# Autodesk Inventor assembly: Wheel_MIR
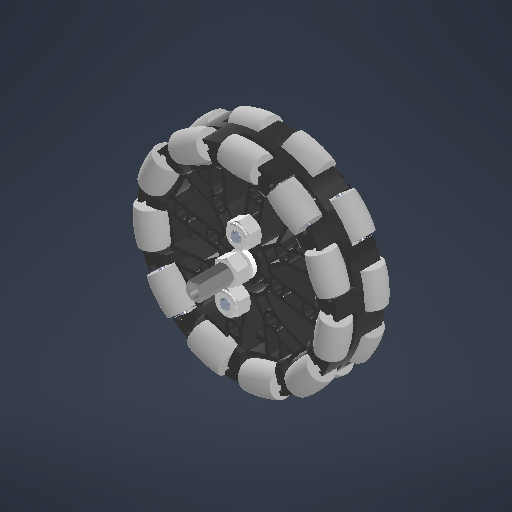
[picture p0: Inventor's stored thumbnail of the model, 512x512]
Saved by Autodesk Inventor 2026.1 (Build 301233000, 233)
## iProperties
Created: 2025-08-03
Part Number: Wheel_MIR
Document SubType Name: Assembly
Designer: roejo
Author: roejo
## Documents named in this file (12)
- C:\Users\roejo\OneDrive\Documents\2026WorldChampionRobot\Robots\Worlds\Subassemblies\Wheel_MIR.iam
- C:\Users\roejo\OneDrive\Documents\2026WorldChampionRobot\Library\Custom Parts\HS 48T Gear, No Insert, Lathe_MIR.iam
- C:\Users\roejo\OneDrive\Documents\2026WorldChampionRobot\Library\VEX-CAD-Inventor-1.4.2\Motion\Spacers\Washer Teflon\TWasher .375 OD x .06250.ipt
- C:\Users\roejo\OneDrive\Documents\2026WorldChampionRobot\Library\VEX-CAD-Inventor-1.4.2\Motion\Spacers\Washer Teflon.ipt
- C:\Users\roejo\OneDrive\Documents\2026WorldChampionRobot\Library\VEX-CAD-Inventor-1.4.2\Structure\Hardware\alu_nylock_MIR.ipt
- C:\Users\roejo\OneDrive\Documents\2026WorldChampionRobot\Library\VEX-CAD-Inventor-1.4.2\Structure\Standoff\Standoff .50.ipt
- C:\Users\roejo\OneDrive\Documents\2026WorldChampionRobot\Library\VEX-CAD-Inventor-1.4.2\Structure\Standoff.ipt
- C:\Users\roejo\OneDrive\Documents\2026WorldChampionRobot\Library\VEX-CAD-Inventor-1.4.2\Structure\Hardware\Screw Steel - Star\SScrew Star Smooth 1.250.ipt
- C:\Users\roejo\OneDrive\Documents\2026WorldChampionRobot\Library\VEX-CAD-Inventor-1.4.2\Structure\Hardware\Screw Steel - Star.ipt
- C:\Users\roejo\OneDrive\Documents\2026WorldChampionRobot\Library\VEX-CAD-Inventor-1.4.2\Motion\Wheels\Omni Wheel\3.25 Omni AS, No Insert_MIR.iam
- C:\Users\roejo\OneDrive\Documents\2026WorldChampionRobot\Library\VEX-CAD-Inventor-1.4.2\Structure\Hardware\Nut Nylon\Nut Nylon - Black.ipt
- C:\Users\roejo\OneDrive\Documents\2026WorldChampionRobot\Library\VEX-CAD-Inventor-1.4.2\Structure\Hardware\Nut Nylon.ipt
## Components (10 placed, 7 different names)
1. HS 48T Gear, No Insert, Lathe_MIR:1 [sub-assembly] — Insert:11, Insert:13, Insert:15, Insert:14, Insert:11
2. TWasher .375 OD x .06250:1 — Insert:5, Insert:18
3. alu_nylock_MIR:1 — Insert:5, Insert:6
4. Standoff .50:1 — Insert:6
5. alu_nylock_MIR:2 — Insert:17
6. SScrew Star Smooth 1.250:1 — Insert:11
7. alu_nylock_MIR:3 — Insert:16
8. SScrew Star Smooth 1.250:2 — Insert:13
9. 3.25 Omni AS, No Insert_MIR:1 [sub-assembly] — Insert:18, Insert:17, Insert:16, Insert:15, Insert:14
10. Nut Nylon - Black:1 — Insert:11
## Relationships (10: Insert 10)
- Insert:5: TWasher .375 OD x .06250:1 ↔ alu_nylock_MIR:1
- Insert:6: alu_nylock_MIR:1 ↔ Standoff .50:1
- Insert:11: HS 48T Gear, No Insert, Lathe_MIR:1 ↔ SScrew Star Smooth 1.250:1
- Insert:13: HS 48T Gear, No Insert, Lathe_MIR:1 ↔ SScrew Star Smooth 1.250:2
- Insert:18: TWasher .375 OD x .06250:1 ↔ 3.25 Omni AS, No Insert_MIR:1
- Insert:17: alu_nylock_MIR:2 ↔ 3.25 Omni AS, No Insert_MIR:1
- Insert:16: alu_nylock_MIR:3 ↔ 3.25 Omni AS, No Insert_MIR:1
- Insert:15: HS 48T Gear, No Insert, Lathe_MIR:1 ↔ 3.25 Omni AS, No Insert_MIR:1
- Insert:14: HS 48T Gear, No Insert, Lathe_MIR:1 ↔ 3.25 Omni AS, No Insert_MIR:1
- Insert:11: HS 48T Gear, No Insert, Lathe_MIR:1 ↔ Nut Nylon - Black:1
